# Autodesk Inventor assembly: hinge asembaly (new)
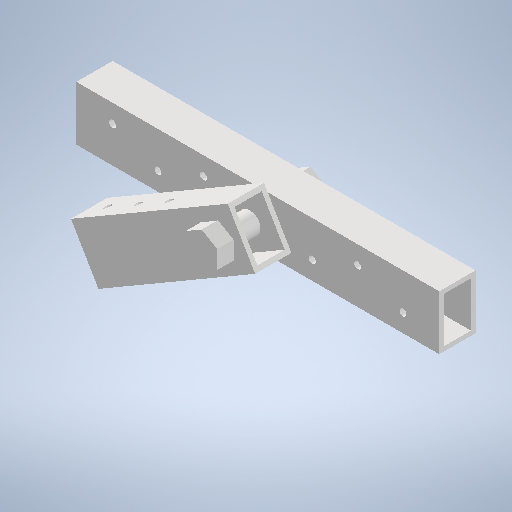
[picture p0: Inventor's stored thumbnail of the model, 512x512]
Saved by Autodesk Inventor 2025.2 (Build 292293000, 293)
## iProperties
Created: 2025-01-08
Part Number: hinge asembaly (new)
Document SubType Name: Assembly
Designer: 5013908
Author: 5013908
## Documents named in this file (4)
- C:\Users\5013908\Documents\GitHub\Mechanical\SeattleSolarCar2024-2025\Frame\hinge asembaly (new).iam
- C:\Users\5013908\Downloads\chassis hinge base.ipt
- C:\Users\5013908\Downloads\canopy hinge part.ipt
- C:\Users\5013908\Downloads\canopy side hinge.ipt
## Components (3 placed, 3 different names)
1. chassis hinge base:1 — Rotational:1
2. canopy hinge part:1 — Flush:1, Rotational:1, Rotational:2
3. canopy side hinge:1 — Flush:2, Rotational:2
## Relationships (4: Flush 2, RevoluteJoint 2)
- Flush:1: canopy hinge part:1
- Rotational:1 [RevoluteJoint]: chassis hinge base:1 ↔ canopy hinge part:1
- Flush:2: canopy side hinge:1
- Rotational:2 [RevoluteJoint]: canopy hinge part:1 ↔ canopy side hinge:1
